# Autodesk Inventor assembly: UNLHEP-14-01-A-001_BonderChuckWplate
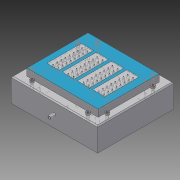
[picture p0: Inventor's stored thumbnail of the model, 180x180]
Saved by Autodesk Inventor 2013 (Build 170138000, 138)
## iProperties
Created: 2014-01-13
Part Number: UNLHEP-14-01-A-001_BonderChuckWplate
Document SubType Name: Assembly
Designer: Frank Meier
Project: UNL Pixel Phase I
Author: Frank Meier
## Documents named in this file (6)
- C:\Users\Frank Meier\Documents\Inventor\Delvotec-Saugplatte\UNLHEP-14-01-A-001_BonderChuckWplate.iam
- C:\Users\Frank Meier\Documents\Inventor\Delvotec-Saugplatte\UNLHEP-14-01-P-002_ChuckForBonder.ipt
- C:\Users\Frank Meier\Documents\Inventor\Delvotec-Saugplatte\UNLHEP-14-01-P-001_ModuleChuck.ipt
- C:\Users\Frank Meier\Documents\Inventor\Delvotec-Saugplatte\UNLHEP-14-01-P-003_Tube4mmID20mm.ipt
- C:\Users\Frank Meier\Documents\Inventor\Content Center Files\R2013\de-DE\ISO 4762(2)\ISO 4762 - M4 x 6ISO.ipt
- C:\Users\Frank Meier\Documents\Inventor\Delvotec-Saugplatte\UNLHEP-14-01-P-005_ModuleStencil.ipt
## Components (12 placed, 5 different names)
1. UNLHEP-14-P-01-002_ChuckForBonder:1 — Passend:1, Passend:2, Einfügen:1, Einfügen:2, Einfügen:3, Einfügen:4, Einfügen:5, Einfügen:6, Einfügen:7, Einfügen:8, Passend:3
2. UNLHEP-14-P-01-001_ModuleChuck:1 — Passend:3, Passend:4, Passend:5, Passend:6, Passend:7, Passend:8, Passend:9
3. UNLHEP-14-01-P-003_Tube4mmID20mm:1 — Passend:1, Passend:2
4. ISO 4762 M4 x 6:1 — Einfügen:1
5. ISO 4762 M4 x 6:2 — Einfügen:2
6. ISO 4762 M4 x 6:3 — Einfügen:3, Passend:4
7. ISO 4762 M4 x 6:4 — Einfügen:4, Passend:5
8. ISO 4762 M4 x 6:5 — Einfügen:5, Passend:6
9. ISO 4762 M4 x 6:6 — Einfügen:6
10. ISO 4762 M4 x 6:7 — Einfügen:7
11. ISO 4762 M4 x 6:8 — Einfügen:8
12. UNLHEP-14-01-P-005_ModuleStencil:1 — Passend:7, Passend:8, Passend:9
## Relationships (17: Mate 9, Insert 8)
- Passend:1 [Mate]: UNLHEP-14-P-01-002_ChuckForBonder:1 ↔ UNLHEP-14-01-P-003_Tube4mmID20mm:1
- Passend:2 [Mate]: UNLHEP-14-P-01-002_ChuckForBonder:1 ↔ UNLHEP-14-01-P-003_Tube4mmID20mm:1
- Passend:3 [Mate]: UNLHEP-14-P-01-002_ChuckForBonder:1 ↔ UNLHEP-14-P-01-001_ModuleChuck:1
- Passend:4 [Mate] (3.5 mm): UNLHEP-14-P-01-001_ModuleChuck:1 ↔ ISO 4762 M4 x 6:3
- Passend:5 [Mate] (3.5 mm): UNLHEP-14-P-01-001_ModuleChuck:1 ↔ ISO 4762 M4 x 6:4
- Passend:6 [Mate] (3.5 mm): UNLHEP-14-P-01-001_ModuleChuck:1 ↔ ISO 4762 M4 x 6:5
- Passend:7 [Mate]: UNLHEP-14-P-01-001_ModuleChuck:1 ↔ UNLHEP-14-01-P-005_ModuleStencil:1
- Passend:8 [Mate]: UNLHEP-14-P-01-001_ModuleChuck:1 ↔ UNLHEP-14-01-P-005_ModuleStencil:1
- Passend:9 [Mate]: UNLHEP-14-P-01-001_ModuleChuck:1 ↔ UNLHEP-14-01-P-005_ModuleStencil:1
- Einfügen:1 [Insert]: UNLHEP-14-P-01-002_ChuckForBonder:1 ↔ ISO 4762 M4 x 6:1
- Einfügen:2 [Insert]: UNLHEP-14-P-01-002_ChuckForBonder:1 ↔ ISO 4762 M4 x 6:2
- Einfügen:3 [Insert]: UNLHEP-14-P-01-002_ChuckForBonder:1 ↔ ISO 4762 M4 x 6:3
- Einfügen:4 [Insert]: UNLHEP-14-P-01-002_ChuckForBonder:1 ↔ ISO 4762 M4 x 6:4
- Einfügen:5 [Insert]: UNLHEP-14-P-01-002_ChuckForBonder:1 ↔ ISO 4762 M4 x 6:5
- Einfügen:6 [Insert]: UNLHEP-14-P-01-002_ChuckForBonder:1 ↔ ISO 4762 M4 x 6:6
- Einfügen:7 [Insert]: UNLHEP-14-P-01-002_ChuckForBonder:1 ↔ ISO 4762 M4 x 6:7
- Einfügen:8 [Insert]: UNLHEP-14-P-01-002_ChuckForBonder:1 ↔ ISO 4762 M4 x 6:8
